# Autodesk Inventor assembly: LiftPrototypeMKI
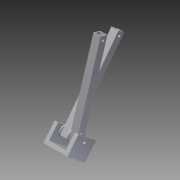
[picture p0: Inventor's stored thumbnail of the model, 180x180]
Saved by Autodesk Inventor 2013 (Build 170138000, 138)
## iProperties
Created: 2013-10-02
Part Number: LiftPrototypeMKI
Document SubType Name: Assembly
Designer: cobrooks
Author: cobrooks
## Documents named in this file (13)
- C:\Users\cobrooks\Documents\GitHub\2013-2014_BlockParty\CAD\Lift\LiftPrototype\LiftPrototypeMKI.iam
- C:\Users\cobrooks\Documents\GitHub\2013-2014_BlockParty\CAD\COTSParts\Structural\5x5mm Box Aluminum.ipt
- C:\Users\cobrooks\Documents\GitHub\2013-2014_BlockParty\CAD\COTSParts\Fasteners\14-20 Washer - Flat.ipt
- C:\Users\cobrooks\Documents\GitHub\2013-2014_BlockParty\CAD\COTSParts\Fasteners\8-32 BHCS x1500.ipt
- C:\Users\cobrooks\Documents\GitHub\2013-2014_BlockParty\CAD\COTSParts\Fasteners\8-32 locknut.ipt
- C:\Users\cobrooks\Documents\GitHub\2013-2014_BlockParty\CAD\COTSParts\Structural\ShortBox.ipt
- C:\Users\cobrooks\Documents\GitHub\2013-2014_BlockParty\CAD\COTSParts\Bosch Extrusion\Bosch 20x40.ipt
- C:\Users\cobrooks\Documents\GitHub\2013-2014_BlockParty\CAD\Lift\LiftPrototype\LiftBase2.ipt
- C:\Users\cobrooks\Documents\GitHub\2013-2014_BlockParty\CAD\COTSParts\Fasteners\8-32 BHCS x2000.ipt
- C:\Users\cobrooks\Documents\GitHub\2013-2014_BlockParty\CAD\Lift\LiftPrototype\ScrewShaft.ipt
- C:\Users\cobrooks\Documents\GitHub\2013-2014_BlockParty\CAD\Lift\LiftPrototype\MotorMount.ipt
- C:\Users\cobrooks\Documents\GitHub\2013-2014_BlockParty\CAD\COTSParts\Tetrix\Hex standoff 1in.ipt
- C:\Users\cobrooks\Documents\GitHub\2013-2014_BlockParty\CAD\Lift\LiftPrototype\Bosch 20x20 Lift slot.ipt
## Components (33 placed, 12 different names)
1. 14-20 Washer - Flat:1 — Insert:2, Insert:3
2. 5x5mm Box Aluminum:1 — Insert:1, Insert:2, Insert:12, Insert:15, Insert:43, Insert:47
3. 5x5mm Box Aluminum:2 — Insert:3, Insert:4, Insert:11, Insert:16, Insert:50
4. 8-32 BHCS x1500:1 — Insert:1
5. 8-32 locknut:1 — Insert:4
6. 5x5mm Box Aluminum:3 — Insert:5, Insert:6, Insert:9, Insert:13
7. 5x5mm Box Aluminum:4 — Insert:7, Insert:8, Insert:10, Insert:14
8. 8-32 BHCS x1500:2 — Insert:5
9. 8-32 locknut:2 — Insert:8
10. 14-20 Washer - Flat:3 — Insert:6, Insert:7
11. 8-32 locknut:3
12. 14-20 Washer - Flat:5 — Insert:9, Insert:12
13. 14-20 Washer - Flat:6 — Insert:10, Insert:11
14. 8-32 BHCS x1500:4 — Insert:13
15. 8-32 BHCS x1500:5 — Insert:14
16. 8-32 locknut:4 — Insert:15
17. 8-32 locknut:5 — Insert:16
18. ShortBox:1 — Insert:25, Insert:27, Insert:49, Angle:2
19. ShortBox:2 — Insert:51, Insert:52, Angle:2
20. 8-32 locknut:6 — Insert:43
21. 14-20 Washer - Flat:8 — Insert:25, Insert:52
22. Bosch 20x40:1 — Mate:10, Flush:1, Flush:2, Mate:11, Mate:12
23. LiftBase2:2 — Insert:29, Insert:30, Insert:31, Mate:10, Flush:1, Flush:2, Insert:53
24. 14-20 Washer - Flat:11 — Insert:27, Insert:29
25. 8-32 BHCS x2000:1 — Insert:30
26. 8-32 locknut:8 — Insert:31
27. ScrewShaft:2
28. Hex standoff 1in:4
29. ScrewShaft:4
30. MotorMount:1 — Insert:47, Insert:51
31. MotorMount:2 — Insert:49, Insert:50
32. Bosch 20x20 Lift slot:1 — Mate:11, Mate:12
33. 14-20 Washer - Flat:12 — Insert:53
## Relationships (34: Insert 28, Mate 3, Flush 2, Angle 1)
- Insert:1: 5x5mm Box Aluminum:1 ↔ 8-32 BHCS x1500:1
- Insert:2: 14-20 Washer - Flat:1 ↔ 5x5mm Box Aluminum:1
- Insert:3: 14-20 Washer - Flat:1 ↔ 5x5mm Box Aluminum:2
- Insert:4: 5x5mm Box Aluminum:2 ↔ 8-32 locknut:1
- Insert:5: 5x5mm Box Aluminum:3 ↔ 8-32 BHCS x1500:2
- Insert:6: 5x5mm Box Aluminum:3 ↔ 14-20 Washer - Flat:3
- Insert:7: 5x5mm Box Aluminum:4 ↔ 14-20 Washer - Flat:3
- Insert:8: 5x5mm Box Aluminum:4 ↔ 8-32 locknut:2
- Insert:9: 5x5mm Box Aluminum:3 ↔ 14-20 Washer - Flat:5
- Insert:10: 5x5mm Box Aluminum:4 ↔ 14-20 Washer - Flat:6
- Insert:11: 5x5mm Box Aluminum:2 ↔ 14-20 Washer - Flat:6
- Insert:12: 5x5mm Box Aluminum:1 ↔ 14-20 Washer - Flat:5
- Insert:13: 5x5mm Box Aluminum:3 ↔ 8-32 BHCS x1500:4
- Insert:14: 5x5mm Box Aluminum:4 ↔ 8-32 BHCS x1500:5
- Insert:15: 5x5mm Box Aluminum:1 ↔ 8-32 locknut:4
- Insert:16: 5x5mm Box Aluminum:2 ↔ 8-32 locknut:5
- Insert:25: ShortBox:1 ↔ 14-20 Washer - Flat:8
- Insert:27: ShortBox:1 ↔ 14-20 Washer - Flat:11
- Insert:29: LiftBase2:2 ↔ 14-20 Washer - Flat:11
- Insert:30: LiftBase2:2 ↔ 8-32 BHCS x2000:1
- Insert:31: LiftBase2:2 ↔ 8-32 locknut:8
- Insert:43: 5x5mm Box Aluminum:1 ↔ 8-32 locknut:6
- Insert:47: 5x5mm Box Aluminum:1 ↔ MotorMount:1
- Insert:49: ShortBox:1 ↔ MotorMount:2
- Insert:50: 5x5mm Box Aluminum:2 ↔ MotorMount:2
- Insert:51: ShortBox:2 ↔ MotorMount:1
- Mate:10: Bosch 20x40:1 ↔ LiftBase2:2
- Flush:1: Bosch 20x40:1 ↔ LiftBase2:2
- Flush:2: Bosch 20x40:1 ↔ LiftBase2:2
- Insert:52: ShortBox:2 ↔ 14-20 Washer - Flat:8
- Angle:2 (20 deg): ShortBox:1 ↔ ShortBox:2
- Mate:11: Bosch 20x40:1 ↔ Bosch 20x20 Lift slot:1
- Mate:12: Bosch 20x40:1 ↔ Bosch 20x20 Lift slot:1
- Insert:53: LiftBase2:2 ↔ 14-20 Washer - Flat:12
